# Autodesk Inventor assembly: transmission with brackets
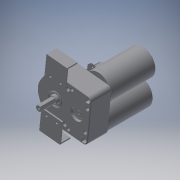
[picture p0: Inventor's stored thumbnail of the model, 180x180]
Saved by Autodesk Inventor 2016 SP2 (Build 200236200, 236)
## iProperties
Created: 2018-01-20
Part Number: transmission with brackets
Document SubType Name: Assembly
Designer: CAD
Author: CAD
## Documents named in this file (3)
- C:\Users\CAD\Documents\GitHub\FIRST-ROBOTICS-2018-5436-CAD\Robot\Chassis\transmission with brackets.iam
- C:\Users\CAD\Documents\GitHub\FIRST-ROBOTICS-2018-5436-CAD\Robot\Chassis\Gutted Transmission (smaller weight on CAD).iam
- C:\Users\CAD\Documents\GitHub\FIRST-ROBOTICS-2018-5436-CAD\Robot\Chassis\improved transmission bracket.ipt
## Components (3 placed, 2 different names)
1. Gutted Transmission (smaller weight on CAD):1 [sub-assembly] — Mate:1, Mate:2, Mate:3, Mate:4, Mate:5, Mate:6
2. improved transmission bracket:1 — Mate:1, Mate:2, Mate:6
3. improved transmission bracket:3 — Mate:3, Mate:4, Mate:5
## Relationships (6: Mate 6)
- Mate:1: Gutted Transmission (smaller weight on CAD):1 ↔ improved transmission bracket:1
- Mate:2: Gutted Transmission (smaller weight on CAD):1 ↔ improved transmission bracket:1
- Mate:3: Gutted Transmission (smaller weight on CAD):1 ↔ improved transmission bracket:3
- Mate:4: Gutted Transmission (smaller weight on CAD):1 ↔ improved transmission bracket:3
- Mate:5: Gutted Transmission (smaller weight on CAD):1 ↔ improved transmission bracket:3
- Mate:6: Gutted Transmission (smaller weight on CAD):1 ↔ improved transmission bracket:1
